# Autodesk Inventor assembly: 607ZZ
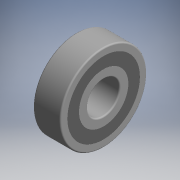
[picture p0: Inventor's stored thumbnail of the model, 180x180]
Saved by Autodesk Inventor 2017.3 (Build 213256000, 256)
## iProperties
Category: PARTsolutions
Company: NTN
Part Number: 607ZZ
Catalog Web Link: www.cadenas.de
Description: With double shield ZZ-
Vendor: NTN
Document SubType Name: Assembly
Designer: partserver
Manufacturer: NTN
Mass: 1.00692 g
Surface Area: 20.317 cm^2
Volume: 1.00692 cm^3
Density: 1 g/cm^3
Title: 607ZZ
Author: Cadenas PARTsolutions
PSOL_IDENT_0: {$CADENAS_DATA\23d-libs\ntn\ball_roller_bearings\miniature_extra_small_bb\metric_system_sizes\mss_zz
PSOL_IDENT_1: _asmtab.prj},182 {VTYP=3D},{STYP=ASSTAB},{NB=607ZZ},{LINA=607ZZ},{NN=With double shield ZZ},{DATE=21
PSOL_IDENT_2: .12.2021 04:23:05},{GEOMDATE=10.03.2020 01:14:46},{VERSION=},{LINEID=12950},{WBVAR=},{WBNUMERIC=}  {
PSOL_IDENT_3: NB=607ZZ},{LINA=607ZZ},{KT=DUMMY},{IDNR=},{SD=7.0},{D=19},{B=6.0},{B1=6.0},{D1=0.0},{D2=0.0},{C1=0.0
PSOL_IDENT_4: },{C2=0.0},{R=0.30},{ORDER=607ZZ},{CR=2480},{COR=910},{CU=60},{CRF=228},{CORF=93},{LSG=34 000},{LSO=
PSOL_IDENT_5: 40 000},{MASS=8.00},{ORDER1=607},{WSS=607ZZ},{WDS=ZZ},{UTWF=0},{FORSS=0},{FORDS=0},{DA1=9},{DA2=10,4
PSOL_IDENT_6: },{DA=17},{RAS=0,3},{MASS1=0.00},{VERS=3},{X=6},{N=7},{O=40.82},{RB=1.776},{PPATH=mss_asmtpl.prj}
NB: 607ZZ
NN: With double shield ZZ
NBSYN: $ORDER.
LINA: 607ZZ
CATALOG: NTN Corporation
SD: 7
D: 19
B1: 6
R: 0.3
ORDER: 607ZZ
CR: 2480
COR: 910
CU: 60
LSG: 34 000
LSO: 40 000
MASS: 8
SUPPLIER: NTN
ARTICLENO: 607ZZ
BOMINFO: 607ZZ
CREATOR: CADENAS GmbH
## Documents named in this file (5)
- e:\temp\worker_31\temp\exporttempdir_6236_156_dlq8i\format_0\607ZZ.iam
- e:\temp\worker_31\temp\exporttempdir_6236_156_dlq8i\format_0\607ZZ Inner ring.ipt
- e:\temp\worker_31\temp\exporttempdir_6236_156_dlq8i\format_0\607ZZ Outer ring.ipt
- e:\temp\worker_31\temp\exporttempdir_6236_156_dlq8i\format_0\607ZZ Shield.ipt
- e:\temp\worker_31\temp\exporttempdir_6236_156_dlq8i\format_0\607ZZ Ball.ipt
## Components (11 placed, 4 different names)
1. 607ZZ Inner ring:1 — mss_ir_Z@1 <-> mss_or_Z@2
2. 607ZZ Outer ring:1 — mss_ir_Z@1 <-> mss_or_Z@2, mss_or_XY@2 <-> mss_s_XY@3, mss_or_Z@2 <-> mss_s_Z@3, mss_or_YZ@2 <-> mss_s_YZ@3, mss_or11_XY@2 <-> mss_s_XY@4, mss_or11_Z@2 <-> mss_s_Z@4, mss_or11_YZ@2 <-> mss_s_YZ@4, mss_or21_1_XY@2 <-> mss_ball_XY@5, mss_or21_1_Z@2 <-> mss_ball_Z@5, mss_or21_1_YZ@2 <-> mss_ball_YZ@5, mss_or21_2_XY@2 <-> mss_ball_XY@6, mss_or21_2_Z@2 <-> mss_ball_Z@6, mss_or21_2_YZ@2 <-> mss_ball_YZ@6, mss_or21_3_XY@2 <-> mss_ball_XY@7, mss_or21_3_Z@2 <-> mss_ball_Z@7, mss_or21_3_YZ@2 <-> mss_ball_YZ@7, mss_or21_4_XY@2 <-> mss_ball_XY@8, mss_or21_4_Z@2 <-> mss_ball_Z@8, mss_or21_4_YZ@2 <-> mss_ball_YZ@8, mss_or21_5_XY@2 <-> mss_ball_XY@9, mss_or21_5_Z@2 <-> mss_ball_Z@9, mss_or21_5_YZ@2 <-> mss_ball_YZ@9, mss_or21_6_XY@2 <-> mss_ball_XY@10, mss_or21_6_Z@2 <-> mss_ball_Z@10, mss_or21_6_YZ@2 <-> mss_ball_YZ@10, mss_or21_7_XY@2 <-> mss_ball_XY@11, mss_or21_7_Z@2 <-> mss_ball_Z@11, mss_or21_7_YZ@2 <-> mss_ball_YZ@11
3. 607ZZ Shield:1 — mss_or_XY@2 <-> mss_s_XY@3, mss_or_Z@2 <-> mss_s_Z@3, mss_or_YZ@2 <-> mss_s_YZ@3
4. 607ZZ Shield:2 — mss_or11_XY@2 <-> mss_s_XY@4, mss_or11_Z@2 <-> mss_s_Z@4, mss_or11_YZ@2 <-> mss_s_YZ@4
5. 607ZZ Ball:1 — mss_or21_1_XY@2 <-> mss_ball_XY@5, mss_or21_1_Z@2 <-> mss_ball_Z@5, mss_or21_1_YZ@2 <-> mss_ball_YZ@5
6. 607ZZ Ball:2 — mss_or21_2_XY@2 <-> mss_ball_XY@6, mss_or21_2_Z@2 <-> mss_ball_Z@6, mss_or21_2_YZ@2 <-> mss_ball_YZ@6
7. 607ZZ Ball:3 — mss_or21_3_XY@2 <-> mss_ball_XY@7, mss_or21_3_Z@2 <-> mss_ball_Z@7, mss_or21_3_YZ@2 <-> mss_ball_YZ@7
8. 607ZZ Ball:4 — mss_or21_4_XY@2 <-> mss_ball_XY@8, mss_or21_4_Z@2 <-> mss_ball_Z@8, mss_or21_4_YZ@2 <-> mss_ball_YZ@8
9. 607ZZ Ball:5 — mss_or21_5_XY@2 <-> mss_ball_XY@9, mss_or21_5_Z@2 <-> mss_ball_Z@9, mss_or21_5_YZ@2 <-> mss_ball_YZ@9
10. 607ZZ Ball:6 — mss_or21_6_XY@2 <-> mss_ball_XY@10, mss_or21_6_Z@2 <-> mss_ball_Z@10, mss_or21_6_YZ@2 <-> mss_ball_YZ@10
11. 607ZZ Ball:7 — mss_or21_7_XY@2 <-> mss_ball_XY@11, mss_or21_7_Z@2 <-> mss_ball_Z@11, mss_or21_7_YZ@2 <-> mss_ball_YZ@11
## Relationships (28: Mate 18, Angle 9, Flush 1)
- mss_ir_Z@1 <-> mss_or_Z@2 [Mate]: 607ZZ Inner ring:1 ↔ 607ZZ Outer ring:1
- mss_or_XY@2 <-> mss_s_XY@3 [Mate]: 607ZZ Outer ring:1 ↔ 607ZZ Shield:1
- mss_or_Z@2 <-> mss_s_Z@3 [Mate]: 607ZZ Outer ring:1 ↔ 607ZZ Shield:1
- mss_or_YZ@2 <-> mss_s_YZ@3 [Angle] (0 deg): 607ZZ Outer ring:1 ↔ 607ZZ Shield:1
- mss_or11_XY@2 <-> mss_s_XY@4 [Flush]: 607ZZ Outer ring:1 ↔ 607ZZ Shield:2
- mss_or11_Z@2 <-> mss_s_Z@4 [Mate]: 607ZZ Outer ring:1 ↔ 607ZZ Shield:2
- mss_or11_YZ@2 <-> mss_s_YZ@4 [Angle] (0 deg): 607ZZ Outer ring:1 ↔ 607ZZ Shield:2
- mss_or21_1_XY@2 <-> mss_ball_XY@5 [Mate]: 607ZZ Outer ring:1 ↔ 607ZZ Ball:1
- mss_or21_1_Z@2 <-> mss_ball_Z@5 [Mate]: 607ZZ Outer ring:1 ↔ 607ZZ Ball:1
- mss_or21_1_YZ@2 <-> mss_ball_YZ@5 [Angle] (0 deg): 607ZZ Outer ring:1 ↔ 607ZZ Ball:1
- mss_or21_2_XY@2 <-> mss_ball_XY@6 [Mate]: 607ZZ Outer ring:1 ↔ 607ZZ Ball:2
- mss_or21_2_Z@2 <-> mss_ball_Z@6 [Mate]: 607ZZ Outer ring:1 ↔ 607ZZ Ball:2
- mss_or21_2_YZ@2 <-> mss_ball_YZ@6 [Angle] (0 deg): 607ZZ Outer ring:1 ↔ 607ZZ Ball:2
- mss_or21_3_XY@2 <-> mss_ball_XY@7 [Mate]: 607ZZ Outer ring:1 ↔ 607ZZ Ball:3
- mss_or21_3_Z@2 <-> mss_ball_Z@7 [Mate]: 607ZZ Outer ring:1 ↔ 607ZZ Ball:3
- mss_or21_3_YZ@2 <-> mss_ball_YZ@7 [Angle] (0 deg): 607ZZ Outer ring:1 ↔ 607ZZ Ball:3
- mss_or21_4_XY@2 <-> mss_ball_XY@8 [Mate]: 607ZZ Outer ring:1 ↔ 607ZZ Ball:4
- mss_or21_4_Z@2 <-> mss_ball_Z@8 [Mate]: 607ZZ Outer ring:1 ↔ 607ZZ Ball:4
- mss_or21_4_YZ@2 <-> mss_ball_YZ@8 [Angle] (0 deg): 607ZZ Outer ring:1 ↔ 607ZZ Ball:4
- mss_or21_5_XY@2 <-> mss_ball_XY@9 [Mate]: 607ZZ Outer ring:1 ↔ 607ZZ Ball:5
- mss_or21_5_Z@2 <-> mss_ball_Z@9 [Mate]: 607ZZ Outer ring:1 ↔ 607ZZ Ball:5
- mss_or21_5_YZ@2 <-> mss_ball_YZ@9 [Angle] (0 deg): 607ZZ Outer ring:1 ↔ 607ZZ Ball:5
- mss_or21_6_XY@2 <-> mss_ball_XY@10 [Mate]: 607ZZ Outer ring:1 ↔ 607ZZ Ball:6
- mss_or21_6_Z@2 <-> mss_ball_Z@10 [Mate]: 607ZZ Outer ring:1 ↔ 607ZZ Ball:6
- mss_or21_6_YZ@2 <-> mss_ball_YZ@10 [Angle] (0 deg): 607ZZ Outer ring:1 ↔ 607ZZ Ball:6
- mss_or21_7_XY@2 <-> mss_ball_XY@11 [Mate]: 607ZZ Outer ring:1 ↔ 607ZZ Ball:7
- mss_or21_7_Z@2 <-> mss_ball_Z@11 [Mate]: 607ZZ Outer ring:1 ↔ 607ZZ Ball:7
- mss_or21_7_YZ@2 <-> mss_ball_YZ@11 [Angle] (0 deg): 607ZZ Outer ring:1 ↔ 607ZZ Ball:7
